# Autodesk Inventor assembly: Lampenkopf_Thumbloop
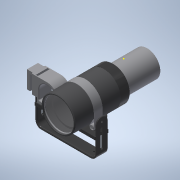
[picture p0: Inventor's stored thumbnail of the model, 180x180]
Saved by Autodesk Inventor 2022 (Build 260153000, 153)
## iProperties
Created: 2014-03-25
Part Number: Lampenkopf_Thumbloop
Document SubType Name: Assembly
Designer: schardt
Author: schardt
## Documents named in this file (15)
- Z:\g.schardt\Inventor\Tauchlampe\Lampenkopf.iam
- Z:\g.schardt\Inventor\Tauchlampe\Haltegriff.ipt
- Z:\g.schardt\Inventor\Tauchlampe\GrundplatteeThumbloop.ipt
- Z:\g.schardt\Inventor\Tauchlampe\Halteblech.ipt
- Z:\g.schardt\Inventor\Tauchlampe\Tools\Thumbloop\LoopD.ipt
- Z:\g.schardt\Inventor\Tauchlampe\Langmutter.ipt
- C:\Users\g.schardt\Documents\Inventor\Content Center Files\R2020\de-DE\ISO 10642(2)\ISO 10642  - M4  x  16.ipt
- C:\Users\g.schardt\Documents\Inventor\Content Center Files\R2020\de-DE\ISO 10642(2)\ISO 10642  - M4  x  10.ipt
- C:\Users\g.schardt\Documents\Inventor\Content Center Files\R2020\de-DE\DIN 976-1 A\DIN 976-1 - M3 x 10 - A.ipt
- C:\Users\g.schardt\Documents\Inventor\Content Center Files\R2020\de-DE\IS 3460 A _ B\IS 3460 - M3 B.ipt
- Z:\g.schardt\Inventor\Tauchlampe\batteriefach_komplett.iam
- Z:\g.schardt\Inventor\Tauchlampe\Überwurfmutter.ipt
- Z:\g.schardt\Inventor\Tauchlampe\Lampengehäuse.iam
- Z:\g.schardt\Inventor\Tauchlampe\O-Ring_53_2_5.ipt
- Z:\g.schardt\Inventor\Tauchlampe\akkufach.ipt
## Components (18 placed, 14 different names)
1. GrundplatteeThumbloop:1 — Passend:1, Passend:2, Fluchtend:2, Passend:11, Passend:12, Passend:13, Passend:37, Tangential:1, Passend:38, Passend:44, Passend:45, Passend:46, Passend:47, Passend:48, Passend:51
2. Haltegriff:1 — Passend:11, Passend:12, Passend:13, Passend:43, Fluchtend:3, Fluchtend:4, Passend:52, Passend:53
3. Lampengehäuse:1 [sub-assembly] — Passend:37, Tangential:1, Passend:38, Einfügen:1, Passend:57, Passend:58, Passend:59, Passend:60, Starr:1, Passend:61, Passend:62, Passend:63
4. Halteblech:1 — Einfügen:1, Passend:39, Passend:40, Passend:41, Passend:42
5. LoopD:1 — Passend:43, Passend:44
6. Langmutter:1 — Passend:39, Passend:40
7. Langmutter:2 — Passend:41, Passend:42
8. DIN EN ISO 10642 M4  x  16:1 — Passend:45
9. DIN EN ISO 10642 M4  x  16:2 — Passend:46
10. DIN EN ISO 10642 M4  x  10:1 — Passend:47
11. DIN 976-1 A M3 x 10:1 — Passend:48, Fluchtend:3, Passend:49
12. IS 3460 A \ B M3 B:1 — Passend:49, Passend:52
13. DIN 976-1 A M3 x 10:2 — Passend:51, Fluchtend:4, Passend:54
14. IS 3460 A \ B M3 B:2 — Passend:53, Passend:54
15. batteriefach_komplett:1 [sub-assembly] — Passend:59, Passend:63
16. Überwurfmutter:1 — Passend:57, Passend:58
17. O-Ring_53_2_5:1 — Passend:60, Starr:1
18. akkufach:1 — Passend:61, Passend:62
## Relationships (35: Mate 29, Flush 3, Tangent 1, Insert 1, WeldJoint 1)
- Passend:1 [Mate]: GrundplatteeThumbloop:1
- Passend:2 [Mate]: GrundplatteeThumbloop:1
- Fluchtend:2 [Flush] (-51 mm): GrundplatteeThumbloop:1
- Passend:11 [Mate]: GrundplatteeThumbloop:1 ↔ Haltegriff:1
- Passend:12 [Mate]: GrundplatteeThumbloop:1 ↔ Haltegriff:1
- Passend:13 [Mate] (30 mm): GrundplatteeThumbloop:1 ↔ Haltegriff:1
- Passend:37 [Mate] (5.5 mm): GrundplatteeThumbloop:1 ↔ Lampengehäuse:1
- Tangential:1: GrundplatteeThumbloop:1 ↔ Lampengehäuse:1
- Passend:38 [Mate] (-5 mm): GrundplatteeThumbloop:1 ↔ Lampengehäuse:1
- Einfügen:1 [Insert] (0.5 mm): Lampengehäuse:1 ↔ Halteblech:1
- Passend:39 [Mate]: Halteblech:1 ↔ Langmutter:1
- Passend:40 [Mate]: Halteblech:1 ↔ Langmutter:1
- Passend:41 [Mate]: Halteblech:1 ↔ Langmutter:2
- Passend:42 [Mate]: Halteblech:1 ↔ Langmutter:2
- Passend:43 [Mate]: Haltegriff:1 ↔ LoopD:1
- Passend:44 [Mate]: GrundplatteeThumbloop:1 ↔ LoopD:1
- Passend:45 [Mate]: GrundplatteeThumbloop:1 ↔ DIN EN ISO 10642 M4  x  16:1
- Passend:46 [Mate]: GrundplatteeThumbloop:1 ↔ DIN EN ISO 10642 M4  x  16:2
- Passend:47 [Mate]: GrundplatteeThumbloop:1 ↔ DIN EN ISO 10642 M4  x  10:1
- Passend:48 [Mate]: GrundplatteeThumbloop:1 ↔ DIN 976-1 A M3 x 10:1
- Fluchtend:3 [Flush] (-2.5 mm): Haltegriff:1 ↔ DIN 976-1 A M3 x 10:1
- Passend:49 [Mate]: DIN 976-1 A M3 x 10:1 ↔ IS 3460 A \ B M3 B:1
- Passend:51 [Mate]: GrundplatteeThumbloop:1 ↔ DIN 976-1 A M3 x 10:2
- Fluchtend:4 [Flush] (-2.5 mm): Haltegriff:1 ↔ DIN 976-1 A M3 x 10:2
- Passend:52 [Mate]: Haltegriff:1 ↔ IS 3460 A \ B M3 B:1
- Passend:53 [Mate]: Haltegriff:1 ↔ IS 3460 A \ B M3 B:2
- Passend:54 [Mate]: DIN 976-1 A M3 x 10:2 ↔ IS 3460 A \ B M3 B:2
- Passend:57 [Mate]: Lampengehäuse:1 ↔ Überwurfmutter:1
- Passend:58 [Mate]: Lampengehäuse:1 ↔ Überwurfmutter:1
- Passend:59 [Mate]: Lampengehäuse:1 ↔ batteriefach_komplett:1
- Passend:60 [Mate]: Lampengehäuse:1 ↔ O-Ring_53_2_5:1
- Starr:1 [WeldJoint] (1.25 mm): Lampengehäuse:1 ↔ O-Ring_53_2_5:1
- Passend:61 [Mate]: Lampengehäuse:1 ↔ akkufach:1
- Passend:62 [Mate]: Lampengehäuse:1 ↔ akkufach:1
- Passend:63 [Mate]: Lampengehäuse:1 ↔ batteriefach_komplett:1
